# Autodesk Inventor assembly: 总2
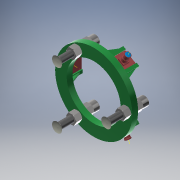
[picture p0: Inventor's stored thumbnail of the model, 180x180]
Saved by Autodesk Inventor 2017 (Build 210142000, 142)
## iProperties
Part Number: 总2
Material: 常规
Document SubType Name: Assembly
Designer: Administrator
Author: Administrator
## Documents named in this file (7)
- D:\大四上\传感器\小轿车\总2.iam
- D:\大四上\传感器\小轿车\支座2.ipt
- D:\大四上\传感器\小轿车\相机.ipt
- D:\大四上\传感器\小轿车\镜头.ipt
- C:\Users\Administrator\Documents\Inventor\Content Center Files\R2017\zh-CN\GB_T 6175-2000\螺母 GB_T 6175 M16.ipt
- C:\Users\Administrator\Documents\Inventor\Content Center Files\R2017\zh-CN\GB_T 70.1-2000\螺钉 GB_T 70.1 M16 x 80.ipt
- D:\大四上\传感器\小轿车\吸盘.ipt
## Components (19 placed, 6 different names)
1. 支座2:1 — 配合:7, 配合:8, 配合:9, 配合:10, 配合:11, 配合:12, 配合:13, 配合:14, 配合:15, 插入:1, 插入:2, 插入:3, 插入:4, 插入:5, 插入:6
2. 相机:1 — 配合:1, 配合:2, 配合:7, 配合:8, 配合:9
3. 镜头:1 — 配合:1, 配合:2
4. 相机:2 — 配合:10, 配合:11, 配合:12
5. 镜头:2
6. 相机:3 — 配合:13, 配合:14, 配合:15
7. 镜头:3
8. 螺母 GB/T 6175-2000 M16:1 — 插入:1, 插入:9
9. 螺母 GB/T 6175-2000 M16:2 — 插入:2, 插入:7
10. 螺母 GB/T 6175-2000 M16:3 — 插入:3, 插入:8
11. 螺母 GB/T 6175-2000 M16:4 — 插入:4
12. 螺母 GB/T 6175-2000 M16:5 — 插入:5
13. 螺母 GB/T 6175-2000 M16:6 — 插入:6
14. 螺钉 GB/T 70.1-2000 M16 x 80:1 — 插入:7, 配合:20, 配合:21
15. 螺钉 GB/T 70.1-2000 M16 x 80:2 — 插入:8, 配合:16, 配合:17
16. 螺钉 GB/T 70.1-2000 M16 x 80:3 — 插入:9, 配合:18, 配合:19
17. 吸盘:1 — 配合:16, 配合:17
18. 吸盘:2 — 配合:18, 配合:19
19. 吸盘:3 — 配合:20, 配合:21
## Relationships (30: Mate 21, Insert 9)
- 配合:1 [Mate]: 相机:1 ↔ 镜头:1
- 配合:2 [Mate]: 相机:1 ↔ 镜头:1
- [Mate]: 相机:2 ↔ 镜头:2
- [Mate]: 相机:2 ↔ 镜头:2
- [Mate]: 相机:3 ↔ 镜头:3
- [Mate]: 相机:3 ↔ 镜头:3
- 配合:7 [Mate]: 支座2:1 ↔ 相机:1
- 配合:8 [Mate]: 支座2:1 ↔ 相机:1
- 配合:9 [Mate]: 支座2:1 ↔ 相机:1
- 配合:10 [Mate]: 支座2:1 ↔ 相机:2
- 配合:11 [Mate]: 支座2:1 ↔ 相机:2
- 配合:12 [Mate]: 支座2:1 ↔ 相机:2
- 配合:13 [Mate]: 支座2:1 ↔ 相机:3
- 配合:14 [Mate]: 支座2:1 ↔ 相机:3
- 配合:15 [Mate]: 支座2:1 ↔ 相机:3
- 插入:1 [Insert]: 支座2:1 ↔ 螺母 GB/T 6175-2000 M16:1
- 插入:2 [Insert]: 支座2:1 ↔ 螺母 GB/T 6175-2000 M16:2
- 插入:3 [Insert]: 支座2:1 ↔ 螺母 GB/T 6175-2000 M16:3
- 插入:4 [Insert]: 支座2:1 ↔ 螺母 GB/T 6175-2000 M16:4
- 插入:5 [Insert]: 支座2:1 ↔ 螺母 GB/T 6175-2000 M16:5
- 插入:6 [Insert]: 支座2:1 ↔ 螺母 GB/T 6175-2000 M16:6
- 插入:7 [Insert]: 螺母 GB/T 6175-2000 M16:2 ↔ 螺钉 GB/T 70.1-2000 M16 x 80:1
- 插入:8 [Insert]: 螺母 GB/T 6175-2000 M16:3 ↔ 螺钉 GB/T 70.1-2000 M16 x 80:2
- 插入:9 [Insert]: 螺母 GB/T 6175-2000 M16:1 ↔ 螺钉 GB/T 70.1-2000 M16 x 80:3
- 配合:16 [Mate]: 螺钉 GB/T 70.1-2000 M16 x 80:2 ↔ 吸盘:1
- 配合:17 [Mate]: 螺钉 GB/T 70.1-2000 M16 x 80:2 ↔ 吸盘:1
- 配合:18 [Mate]: 螺钉 GB/T 70.1-2000 M16 x 80:3 ↔ 吸盘:2
- 配合:19 [Mate]: 螺钉 GB/T 70.1-2000 M16 x 80:3 ↔ 吸盘:2
- 配合:20 [Mate]: 螺钉 GB/T 70.1-2000 M16 x 80:1 ↔ 吸盘:3
- 配合:21 [Mate]: 螺钉 GB/T 70.1-2000 M16 x 80:1 ↔ 吸盘:3
## Named parameters: d2_d0 = 0 mm, d3_d1 = 0 mm, d4_d0 = 0 mm, d5_d1 = 0 mm
